# Autodesk Inventor assembly: Z Axis
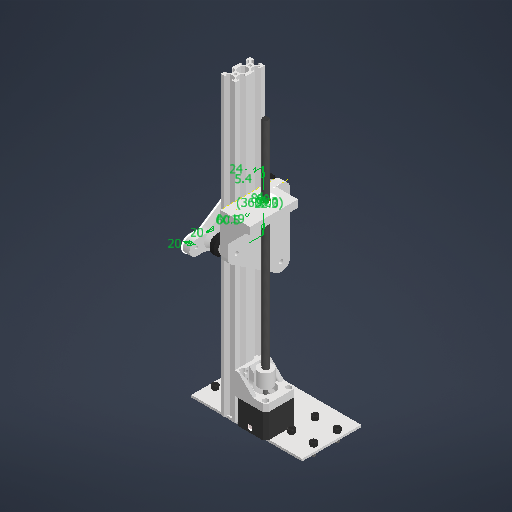
[picture p0: Inventor's stored thumbnail of the model, 512x512]
Saved by Autodesk Inventor 2025.1 (Build 291241000, 241)
## iProperties
Created: 2025-01-21
Part Number: Z Axis
Document SubType Name: Assembly
Designer: jerem
Author: jerem
## Documents named in this file (13)
- C:\Users\jerem\Documents\GitHub\Perovskite-Automated-Synthesis-System\CAD\Gantry\Z Axis.iam
- C:\Users\jerem\Documents\GitHub\Perovskite-Automated-Synthesis-System\CAD\Non 3D Printed Parts\X Axis Base Plate.ipt
- C:\Users\jerem\Documents\GitHub\Perovskite-Automated-Synthesis-System\CAD\Non 3D Printed Parts\Extrusion\V Extrustion 40x400mm.ipt
- C:\Users\jerem\Documents\GitHub\Perovskite-Automated-Synthesis-System\CAD\Non 3D Printed Parts\Screws\M5x12.ipt
- C:\Users\jerem\Documents\GitHub\Perovskite-Automated-Synthesis-System\CAD\Non 3D Printed Parts\Motors and Servos\NEMA17 Stepper Motor.ipt
- C:\Users\jerem\Documents\GitHub\Perovskite-Automated-Synthesis-System\CAD\Non 3D Printed Parts\Threaded Rod 300mm.ipt
- C:\Users\jerem\Documents\GitHub\Perovskite-Automated-Synthesis-System\CAD\Non 3D Printed Parts\Rod Coupler.ipt
- C:\Users\jerem\Documents\GitHub\Perovskite-Automated-Synthesis-System\CAD\Non 3D Printed Parts\Nuts\M4 T-Slot Nut.ipt
- C:\Users\jerem\Documents\GitHub\Perovskite-Automated-Synthesis-System\CAD\Gantry\Part21.ipt
- C:\Users\jerem\Documents\GitHub\Perovskite-Automated-Synthesis-System\CAD\Gantry\y axis something.ipt
- C:\Users\jerem\Documents\GitHub\Perovskite-Automated-Synthesis-System\CAD\Non 3D Printed Parts\Leadscrew.ipt
- C:\Users\jerem\Documents\GitHub\Perovskite-Automated-Synthesis-System\CAD\Non 3D Printed Parts\Printer Wheel.ipt
- C:\Users\jerem\Documents\GitHub\Perovskite-Automated-Synthesis-System\CAD\Gantry\y axis something back.ipt
## Components (22 placed, 12 different names)
1. X Axis Base Plate:1 — Mate:1, Mate:2, Mate:3, Mate:4, Mate:5, Mate:6, Mate:7, Mate:8, Mate:9, Mate:10, Mate:11, Mate:12, Mate:13, Mate:14, Mate:15, Mate:16, Mate:17, Mate:26, Angle:1
2. V Extrustion 40x400mm:1 — Mate:1, Mate:25, Angle:1, Mate:30, Angle:2, Angle:3, Mate:32, Flush:1, Angle:4
3. M5x12:1 — Mate:2, Mate:3
4. M5x12:2 — Mate:4, Mate:17
5. M5x12:3 — Mate:9, Mate:12
6. M5x12:4 — Mate:8, Mate:13
7. M5x12:5 — Mate:7, Mate:15
8. M5x12:6 — Mate:6, Mate:14
9. M5x12:7 — Mate:5, Mate:16
10. M5x12:8 — Mate:10, Mate:11
11. NEMA17 Stepper Motor:1 — Mate:25, Mate:26, Mate:33, Mate:34, Mate:35, Flush:1
12. Threaded Rod 300mm:1 — Mate:41
13. Rod Coupler:1
14. M4 T-Slot Nut:1 — Mate:30, Angle:2, Mate:37
15. M4 T-Slot Nut:2 — Angle:3, Mate:32, Mate:36
16. Part21:1 — Mate:33, Mate:34, Mate:35, Mate:36, Mate:37
17. y axis something:1 — Mate:38, Mate:39, Mate:40, Angle:4, Mate:42, Mate:43, Mate:44, Mate:45, Mate:46, Mate:47
18. Leadscrew:1 — Mate:38, Mate:39, Mate:40, Mate:41
19. Printer Wheel:1 — Mate:43, Mate:45, Symmetry:1
20. Printer Wheel:2 — Mate:44, Mate:47, Symmetry:1, Mate:48
21. Printer Wheel:3 — Mate:42, Mate:46, Mate:49, Mate:50
22. y axis something back:1 — Mate:48, Mate:49, Mate:50
## Relationships (49: Mate 43, Angle 4, Flush 1, Symmetry 1)
- Mate:1: X Axis Base Plate:1 ↔ V Extrustion 40x400mm:1
- Mate:2: X Axis Base Plate:1 ↔ M5x12:1
- Mate:3: X Axis Base Plate:1 ↔ M5x12:1
- Mate:4: X Axis Base Plate:1 ↔ M5x12:2
- Mate:5: X Axis Base Plate:1 ↔ M5x12:7
- Mate:6: X Axis Base Plate:1 ↔ M5x12:6
- Mate:7: X Axis Base Plate:1 ↔ M5x12:5
- Mate:8: X Axis Base Plate:1 ↔ M5x12:4
- Mate:9: X Axis Base Plate:1 ↔ M5x12:3
- Mate:10: X Axis Base Plate:1 ↔ M5x12:8
- Mate:11: X Axis Base Plate:1 ↔ M5x12:8
- Mate:12: X Axis Base Plate:1 ↔ M5x12:3
- Mate:13: X Axis Base Plate:1 ↔ M5x12:4
- Mate:14: X Axis Base Plate:1 ↔ M5x12:6
- Mate:15: X Axis Base Plate:1 ↔ M5x12:5
- Mate:16: X Axis Base Plate:1 ↔ M5x12:7
- Mate:17: X Axis Base Plate:1 ↔ M5x12:2
- [Mate]: NEMA17 Stepper Motor:1 ↔ Rod Coupler:1
- [Mate]: Threaded Rod 300mm:1 ↔ Rod Coupler:1
- [Mate] (-8 mm): NEMA17 Stepper Motor:1 ↔ Rod Coupler:1
- [Mate] (-8 mm): Threaded Rod 300mm:1 ↔ Rod Coupler:1
- Mate:25: V Extrustion 40x400mm:1 ↔ NEMA17 Stepper Motor:1
- Mate:26: X Axis Base Plate:1 ↔ NEMA17 Stepper Motor:1
- Angle:1 (0 deg): X Axis Base Plate:1 ↔ V Extrustion 40x400mm:1
- Mate:30: V Extrustion 40x400mm:1 ↔ M4 T-Slot Nut:1
- Angle:2 (0 deg): V Extrustion 40x400mm:1 ↔ M4 T-Slot Nut:1
- Angle:3 (0 deg): V Extrustion 40x400mm:1 ↔ M4 T-Slot Nut:2
- Mate:32: V Extrustion 40x400mm:1 ↔ M4 T-Slot Nut:2
- Mate:33: NEMA17 Stepper Motor:1 ↔ Part21:1
- Mate:34: NEMA17 Stepper Motor:1 ↔ Part21:1
- Mate:35: NEMA17 Stepper Motor:1 ↔ Part21:1
- Mate:36: M4 T-Slot Nut:2 ↔ Part21:1
- Mate:37: M4 T-Slot Nut:1 ↔ Part21:1
- Flush:1: V Extrustion 40x400mm:1 ↔ NEMA17 Stepper Motor:1
- Mate:38: y axis something:1 ↔ Leadscrew:1
- Mate:39: y axis something:1 ↔ Leadscrew:1
- Mate:40: y axis something:1 ↔ Leadscrew:1
- Mate:41: Threaded Rod 300mm:1 ↔ Leadscrew:1
- Angle:4 (180 deg): V Extrustion 40x400mm:1 ↔ y axis something:1
- Mate:42: y axis something:1 ↔ Printer Wheel:3
- Mate:43: y axis something:1 ↔ Printer Wheel:1
- Mate:44: y axis something:1 ↔ Printer Wheel:2
- Mate:45: y axis something:1 ↔ Printer Wheel:1
- Mate:46: y axis something:1 ↔ Printer Wheel:3
- Mate:47: y axis something:1 ↔ Printer Wheel:2
- Symmetry:1: Printer Wheel:1 ↔ Printer Wheel:2
- Mate:48: Printer Wheel:2 ↔ y axis something back:1
- Mate:49: Printer Wheel:3 ↔ y axis something back:1
- Mate:50: Printer Wheel:3 ↔ y axis something back:1
